# Autodesk Inventor assembly: carrier
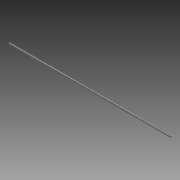
[picture p0: Inventor's stored thumbnail of the model, 180x180]
Saved by Autodesk Inventor 2013 (Build 170138000, 138)
## iProperties
Created: 2013-01-14
Part Number: carrier
Document SubType Name: Assembly
Designer: Istvan
Author: Istvan
## Documents named in this file (2)
- E:\GitHub\Crown-Fire\CAD\Electronics\carrier\carrier.iam
- E:\GitHub\Crown-Fire\CAD\Electronics\carrier\carrierSegment.ipt
## Components (92 placed, 1 different names)
1. carrierSegment:1
2. carrierSegment:2
3. carrierSegment:3
4. carrierSegment:4
5. carrierSegment:5
6. carrierSegment:6
7. carrierSegment:7
8. carrierSegment:8
9. carrierSegment:9
10. carrierSegment:10
11. carrierSegment:11
12. carrierSegment:12
13. carrierSegment:13
14. carrierSegment:14
15. carrierSegment:15
16. carrierSegment:16
17. carrierSegment:17
18. carrierSegment:18
19. carrierSegment:19
20. carrierSegment:20
21. carrierSegment:21
22. carrierSegment:22
23. carrierSegment:23
24. carrierSegment:24
25. carrierSegment:25
26. carrierSegment:26
27. carrierSegment:27
28. carrierSegment:28
29. carrierSegment:29
30. carrierSegment:30
31. carrierSegment:31
32. carrierSegment:32
33. carrierSegment:33
34. carrierSegment:34
35. carrierSegment:35
36. carrierSegment:36
37. carrierSegment:37
38. carrierSegment:38
39. carrierSegment:39
40. carrierSegment:40
41. carrierSegment:41
42. carrierSegment:42
43. carrierSegment:43
44. carrierSegment:44
45. carrierSegment:45
46. carrierSegment:46
47. carrierSegment:47
48. carrierSegment:48
49. carrierSegment:49
50. carrierSegment:50
51. carrierSegment:51
52. carrierSegment:52
53. carrierSegment:53
54. carrierSegment:54
55. carrierSegment:55
56. carrierSegment:56
57. carrierSegment:57
58. carrierSegment:58
59. carrierSegment:59
60. carrierSegment:60
61. carrierSegment:61
62. carrierSegment:62
63. carrierSegment:63
64. carrierSegment:64
65. carrierSegment:65
66. carrierSegment:66
67. carrierSegment:67
68. carrierSegment:68
69. carrierSegment:69
70. carrierSegment:70
71. carrierSegment:71
72. carrierSegment:72
73. carrierSegment:73
74. carrierSegment:74
75. carrierSegment:75
76. carrierSegment:76
77. carrierSegment:77
78. carrierSegment:78
79. carrierSegment:79
80. carrierSegment:80
81. carrierSegment:81
82. carrierSegment:82
83. carrierSegment:83
84. carrierSegment:84
85. carrierSegment:85
86. carrierSegment:86
87. carrierSegment:87
88. carrierSegment:88
89. carrierSegment:89
90. carrierSegment:90
91. carrierSegment:91
92. carrierSegment:92
## Component patterns: (92 elements, first: carrierSegment:1)
